# Autodesk Inventor assembly: remmy
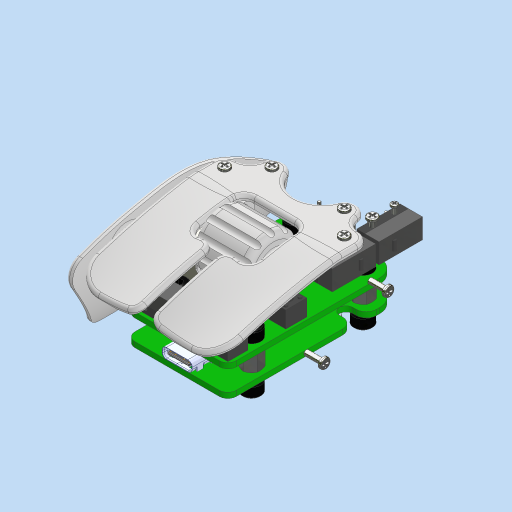
[picture p0: Inventor's stored thumbnail of the model, 512x512]
Saved by Autodesk Inventor 2024 (Build 280153000, 153)
## iProperties
Created: 2025-05-08
Part Number: remmy
Document SubType Name: Assembly
Designer: XxPan
Author: XxPan
## Documents named in this file (12)
- C:\Users\XxPan\OneDrive - McMaster University\Mouse\CAD\remmy.iam
- C:\Users\XxPan\OneDrive - McMaster University\Mouse\CAD\mcu_board.iam
- C:\Users\XxPan\OneDrive - McMaster University\Mouse\CAD\sensor_board.iam
- C:\Users\XxPan\OneDrive - McMaster University\Mouse\CAD\M3_H8.0mm_board_spacer.ipt
- C:\Users\XxPan\OneDrive - McMaster University\Mouse\CAD\socket_head_cap_screw_M3x5.ipt
- C:\Users\XxPan\OneDrive - McMaster University\Mouse\CAD\shell\base_plate.ipt
- C:\Users\XxPan\OneDrive - McMaster University\Mouse\CAD\pan_head_screw_M1.6x5.ipt
- C:\Users\XxPan\OneDrive - McMaster University\Mouse\CAD\pan_head_screw_M1.2x4.ipt
- C:\Users\XxPan\OneDrive - McMaster University\Mouse\CAD\shell\mouse_buttons_1-2.ipt
- C:\Users\XxPan\OneDrive - McMaster University\Mouse\CAD\Atmel-ICE_adapter.ipt
- C:\Users\XxPan\OneDrive - McMaster University\Mouse\CAD\shell\thumb_pad_shortened.ipt
- C:\Users\XxPan\OneDrive - McMaster University\Mouse\CAD\shell\pinky_pad_v2.ipt
## Components (32 placed, 11 different names)
1. mcu_board:1 [sub-assembly] — Mate:5, Flush:1, Flush:2, Insert:5, Insert:6, Insert:7, Insert:8, Mate:8, Flush:6, Flush:7
2. sensor_board:1 [sub-assembly] — Mate:1, Mate:2, Mate:3, Mate:4, Flush:1, Flush:2, Insert:1, Insert:2, Insert:3, Insert:4, Insert:9, Insert:10
3. base_plate:1 — Insert:9, Insert:10, Insert:21, Insert:22, Insert:23, Insert:24, Insert:36, Insert:37, Insert:42, Insert:43, Insert:44, Insert:45
4. Atmel-ICE_adapter:1 — Mate:8, Flush:6, Flush:7
5. thumb_pad_shortened:1 — Insert:36, Insert:37
6. pinky_pad_v2:1 — Insert:42, Insert:43, Insert:50, Insert:51, Insert:52
7. mouse_buttons_1-2:1 — Insert:44, Insert:45, Insert:46, Insert:47, Insert:48, Insert:49
8. M3_H8.0mm_board_spacer:1 — Mate:2, Insert:3
9. M3_H8.0mm_board_spacer:2 — Mate:1, Mate:5, Insert:4
10. M3_H8.0mm_board_spacer:3 — Mate:4, Insert:2
11. M3_H8.0mm_board_spacer:4 — Mate:3, Insert:1
12. socket_head_cap_screw_M3x5:1 — Insert:8
13. socket_head_cap_screw_M3x5:2 — Insert:7
14. socket_head_cap_screw_M3x5:3
15. socket_head_cap_screw_M3x5:4
16. socket_head_cap_screw_M3x5:5
17. socket_head_cap_screw_M3x5:6 — Insert:6
18. socket_head_cap_screw_M3x5:7 — Insert:5
19. socket_head_cap_screw_M3x5:8
20. pan_head_screw_M1.6x5:2
21. pan_head_screw_M1.6x5:3
22. pan_head_screw_M1.6x5:4 — Insert:50
23. pan_head_screw_M1.6x5:5 — Insert:51
24. pan_head_screw_M1.6x5:6 — Insert:52
25. pan_head_screw_M1.6x5:7 — Insert:24
26. pan_head_screw_M1.6x5:8 — Insert:23
27. pan_head_screw_M1.2x4:1 — Insert:22
28. pan_head_screw_M1.2x4:2 — Insert:21
29. pan_head_screw_M1.6x5:9 — Insert:46
30. pan_head_screw_M1.6x5:10 — Insert:48
31. pan_head_screw_M1.6x5:11 — Insert:49
32. pan_head_screw_M1.6x5:12 — Insert:47
## Relationships (37: Insert 27, Mate 6, Flush 4)
- Mate:1: sensor_board:1 ↔ M3_H8.0mm_board_spacer:2
- Mate:2: sensor_board:1 ↔ M3_H8.0mm_board_spacer:1
- Mate:3: sensor_board:1 ↔ M3_H8.0mm_board_spacer:4
- Mate:4: sensor_board:1 ↔ M3_H8.0mm_board_spacer:3
- Mate:5: mcu_board:1 ↔ M3_H8.0mm_board_spacer:2
- Flush:1: mcu_board:1 ↔ sensor_board:1
- Flush:2: mcu_board:1 ↔ sensor_board:1
- Insert:1: sensor_board:1 ↔ M3_H8.0mm_board_spacer:4
- Insert:2: sensor_board:1 ↔ M3_H8.0mm_board_spacer:3
- Insert:3: sensor_board:1 ↔ M3_H8.0mm_board_spacer:1
- Insert:4: sensor_board:1 ↔ M3_H8.0mm_board_spacer:2
- Insert:5: mcu_board:1 ↔ socket_head_cap_screw_M3x5:7
- Insert:6: mcu_board:1 ↔ socket_head_cap_screw_M3x5:6
- Insert:7: mcu_board:1 ↔ socket_head_cap_screw_M3x5:2
- Insert:8: mcu_board:1 ↔ socket_head_cap_screw_M3x5:1
- Insert:9: sensor_board:1 ↔ base_plate:1
- Insert:10: sensor_board:1 ↔ base_plate:1
- Insert:21: base_plate:1 ↔ pan_head_screw_M1.2x4:2
- Insert:22: base_plate:1 ↔ pan_head_screw_M1.2x4:1
- Insert:23: base_plate:1 ↔ pan_head_screw_M1.6x5:8
- Insert:24: base_plate:1 ↔ pan_head_screw_M1.6x5:7
- Mate:8: mcu_board:1 ↔ Atmel-ICE_adapter:1
- Flush:6: mcu_board:1 ↔ Atmel-ICE_adapter:1
- Flush:7: mcu_board:1 ↔ Atmel-ICE_adapter:1
- Insert:36: base_plate:1 ↔ thumb_pad_shortened:1
- Insert:37: base_plate:1 ↔ thumb_pad_shortened:1
- Insert:42: base_plate:1 ↔ pinky_pad_v2:1
- Insert:43: base_plate:1 ↔ pinky_pad_v2:1
- Insert:44: base_plate:1 ↔ mouse_buttons_1-2:1
- Insert:45: base_plate:1 ↔ mouse_buttons_1-2:1
- Insert:46: mouse_buttons_1-2:1 ↔ pan_head_screw_M1.6x5:9
- Insert:47: mouse_buttons_1-2:1 ↔ pan_head_screw_M1.6x5:12
- Insert:48: mouse_buttons_1-2:1 ↔ pan_head_screw_M1.6x5:10
- Insert:49: mouse_buttons_1-2:1 ↔ pan_head_screw_M1.6x5:11
- Insert:50: pinky_pad_v2:1 ↔ pan_head_screw_M1.6x5:4
- Insert:51: pinky_pad_v2:1 ↔ pan_head_screw_M1.6x5:5
- Insert:52: pinky_pad_v2:1 ↔ pan_head_screw_M1.6x5:6
